# Autodesk Inventor assembly: Reducer_Motor_HG-KR53
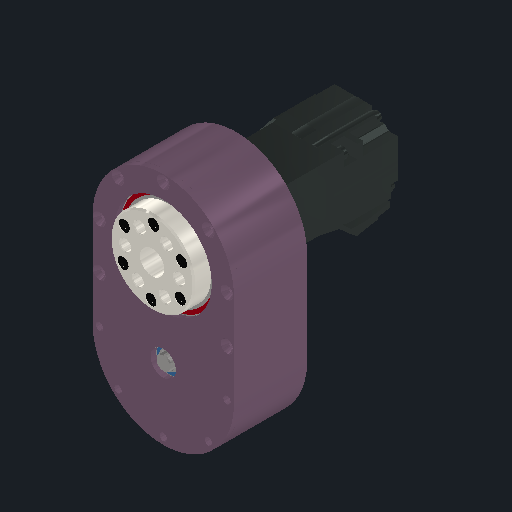
[picture p0: Inventor's stored thumbnail of the model, 512x512]
Saved by Autodesk Inventor 2026 (Build 300175000, 175)
## iProperties
Created: 2025-12-04
Part Number: Reducer_Motor_HG-KR53
Document SubType Name: Assembly
Designer: DanielFGarzon
Mass: 1057.96 g
Surface Area: 1185.99 cm^2
Volume: 274.829 cm^3
Density: 3.84952 g/cm^3
Author: DanielFGarzon
## Documents named in this file (17)
- D:\POLIMI\3RD SEMESTER\Industrial Robotics\Project\Mine\Reducer_02\Reducer_Motor_HG-KR53.iam
- D:\POLIMI\3RD SEMESTER\Industrial Robotics\Project\Mine\Reducer_02\Housing.ipt
- D:\POLIMI\3RD SEMESTER\Industrial Robotics\Project\Mine\Reducer_02\Bearing_08_16_04.ipt
- D:\POLIMI\3RD SEMESTER\Industrial Robotics\Project\Mine\Reducer_02\Bearing_08_26_08.ipt
- D:\POLIMI\3RD SEMESTER\Industrial Robotics\Project\Mine\Reducer_02\Shaft_8mm.ipt
- D:\POLIMI\3RD SEMESTER\Industrial Robotics\Project\Mine\Reducer_02\Washer_M8_12_0.3.ipt
- D:\POLIMI\3RD SEMESTER\Industrial Robotics\Project\Mine\Reducer_02\Pulley_3M12T_01.ipt
- D:\POLIMI\3RD SEMESTER\Industrial Robotics\Project\Mine\Reducer_02\Washer_M8_10_3.8.ipt
- D:\POLIMI\3RD SEMESTER\Industrial Robotics\Project\Mine\Reducer_02\Pulley_3M60T_01.ipt
- D:\POLIMI\3RD SEMESTER\Industrial Robotics\Project\Mine\Reducer_02\Washer_M8_14_0.5.ipt
- D:\POLIMI\3RD SEMESTER\Industrial Robotics\Project\Mine\Reducer_02\Pulley_3M12T_02.ipt
- D:\POLIMI\3RD SEMESTER\Industrial Robotics\Project\Mine\Reducer_02\Pulley_3M60T_02.ipt
- D:\POLIMI\3RD SEMESTER\Industrial Robotics\Project\Mine\Reducer_02\ActuationDisk.ipt
- D:\POLIMI\3RD SEMESTER\Industrial Robotics\Project\Mine\Reducer_02\Bearing_45_55_06.ipt
- D:\POLIMI\3RD SEMESTER\Industrial Robotics\Project\Mine\Reducer_02\Cover.ipt
- D:\POLIMI\3RD SEMESTER\Industrial Robotics\Project\Mine\Reducer_02\Motor_HG-KR053.ipt
- D:\POLIMI\3RD SEMESTER\Industrial Robotics\Project\Mine\Reducer_02\M3_Screw.ipt
## Components (23 placed, 16 different names)
1. Housing:1 — Mate:1, Mate:2, Flush:1, Mate:45, Mate:50, Mate:51, Mate:52
2. Bearing_08_16_04:1 — Mate:1, Mate:2, Mate:3, Mate:7
3. Bearing_08_26_08:1 — Mate:30, Mate:34, Mate:35
4. Shaft_8mm:1 — Mate:3, Flush:1, Mate:8, Mate:20, Mate:27, Mate:32, Mate:47
5. Washer_M8_12_0.3:1 — Mate:7, Mate:8, Mate:26
6. Pulley_3M12T_01:1 — Mate:23, Mate:28
7. Washer_M8_10_3.8:1 — Mate:23
8. Pulley_3M60T_01:1 — Mate:26, Mate:27, Mate:33
9. Washer_M8_14_0.5:1 — Mate:28, Mate:30
10. Washer_M8_14_0.5:2 — Mate:20, Mate:31, Mate:33
11. Pulley_3M12T_02:1 — Mate:31, Mate:32
12. Pulley_3M60T_02:1 — Mate:34, Mate:35, Mate:40, Mate:41, Mate:42
13. ActuationDisk:1 — Mate:40, Mate:41, Mate:42, Mate:43, Mate:44, Mate:46, Mate:53, Mate:54, Mate:55, Mate:56, Mate:57, Mate:58, Flush:2, Flush:3, Flush:4, Flush:5, Flush:6, Flush:7
14. Bearing_45_55_06:1 — Mate:43, Mate:44
15. Cover:1 — Mate:45, Mate:46, Mate:47, Mate:48, Mate:49
16. Bearing_08_16_04:3 — Mate:48, Mate:49
17. Motor_HG-KR053:1 — Mate:50, Mate:51, Mate:52
18. M3_Screw:1 — Mate:54, Flush:3
19. M3_Screw:2 — Mate:55, Flush:4
20. M3_Screw:3 — Mate:56, Flush:5
21. M3_Screw:4 — Mate:58, Flush:7
22. M3_Screw:5 — Mate:57, Flush:6
23. M3_Screw:6 — Mate:53, Flush:2
## Relationships (42: Mate 35, Flush 7)
- Mate:1: Housing:1 ↔ Bearing_08_16_04:1
- Mate:2: Housing:1 ↔ Bearing_08_16_04:1
- Mate:3: Bearing_08_16_04:1 ↔ Shaft_8mm:1
- Flush:1: Housing:1 ↔ Shaft_8mm:1
- Mate:7: Bearing_08_16_04:1 ↔ Washer_M8_12_0.3:1
- Mate:8: Shaft_8mm:1 ↔ Washer_M8_12_0.3:1
- Mate:20: Shaft_8mm:1 ↔ Washer_M8_14_0.5:2
- Mate:23: Pulley_3M12T_01:1 ↔ Washer_M8_10_3.8:1
- Mate:26: Washer_M8_12_0.3:1 ↔ Pulley_3M60T_01:1
- Mate:27: Shaft_8mm:1 ↔ Pulley_3M60T_01:1
- Mate:28: Pulley_3M12T_01:1 ↔ Washer_M8_14_0.5:1
- Mate:30: Bearing_08_26_08:1 ↔ Washer_M8_14_0.5:1
- Mate:31: Washer_M8_14_0.5:2 ↔ Pulley_3M12T_02:1
- Mate:32: Shaft_8mm:1 ↔ Pulley_3M12T_02:1
- Mate:33: Pulley_3M60T_01:1 ↔ Washer_M8_14_0.5:2
- Mate:34: Bearing_08_26_08:1 ↔ Pulley_3M60T_02:1
- Mate:35: Bearing_08_26_08:1 ↔ Pulley_3M60T_02:1
- Mate:40: Pulley_3M60T_02:1 ↔ ActuationDisk:1
- Mate:41: Pulley_3M60T_02:1 ↔ ActuationDisk:1
- Mate:42: Pulley_3M60T_02:1 ↔ ActuationDisk:1
- Mate:43: ActuationDisk:1 ↔ Bearing_45_55_06:1
- Mate:44: ActuationDisk:1 ↔ Bearing_45_55_06:1
- Mate:45: Housing:1 ↔ Cover:1
- Mate:46: ActuationDisk:1 ↔ Cover:1
- Mate:47: Shaft_8mm:1 ↔ Cover:1
- Mate:48: Cover:1 ↔ Bearing_08_16_04:3
- Mate:49: Cover:1 ↔ Bearing_08_16_04:3
- Mate:50: Housing:1 ↔ Motor_HG-KR053:1
- Mate:51: Housing:1 ↔ Motor_HG-KR053:1
- Mate:52: Housing:1 ↔ Motor_HG-KR053:1
- Mate:53: ActuationDisk:1 ↔ M3_Screw:6
- Mate:54: ActuationDisk:1 ↔ M3_Screw:1
- Mate:55: ActuationDisk:1 ↔ M3_Screw:2
- Mate:56: ActuationDisk:1 ↔ M3_Screw:3
- Mate:57: ActuationDisk:1 ↔ M3_Screw:5
- Mate:58: ActuationDisk:1 ↔ M3_Screw:4
- Flush:2: ActuationDisk:1 ↔ M3_Screw:6
- Flush:3: ActuationDisk:1 ↔ M3_Screw:1
- Flush:4: ActuationDisk:1 ↔ M3_Screw:2
- Flush:5: ActuationDisk:1 ↔ M3_Screw:3
- Flush:6: ActuationDisk:1 ↔ M3_Screw:5
- Flush:7: ActuationDisk:1 ↔ M3_Screw:4
